# Autodesk Inventor assembly: SKF_SYWK 30 YTH
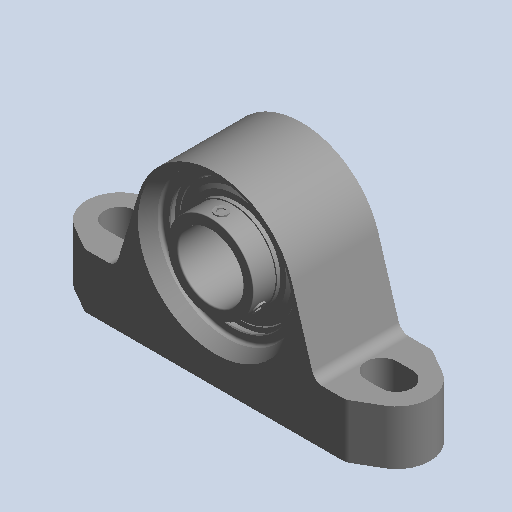
[picture p0: Inventor's stored thumbnail of the model, 512x512]
Saved by Autodesk Inventor 2022.1 (Build 261234000, 234)
## iProperties
Category: PARTsolutions
Company: SKF
Part Number: SKF_SYWK 30 YTH
Catalog Web Link: www.cadenas.de
Description: AYP_001_HC_HH_HY-AYL_001_HP-Y-bearing plummer block units
Vendor: SKF
Document SubType Name: Assembly
Designer: partserver
Manufacturer: SKF
Mass: 431.299 g
Surface Area: 643.844 cm^2
Volume: 166.494 cm^3
Density: 2.59047 g/cm^3
PSOL_IDENT_0: {$CADENAS_DATA\23d-libs\skf\bearings_units_and_housings\bearing_units\ball_bearing_units\y-units\ayp
PSOL_IDENT_1: _001_hc_hh_hy-ayl_001_hp.prj},212 {VTYP=3D},{STYP=ASSTAB},{NB=SKF_SYWK 30 YTH},{LINA=SKF_SYWK 30 YTH
PSOL_IDENT_2: },{NN=AYP_001_HC_HH_HY-AYL_001_HP},{DATE=17.09.2021 07:33:22},{GEOMDATE=07.09.2021 05:49:17},{VERSIO
PSOL_IDENT_3: N=},{LINEID=6610},{WBVAR=COVER},{WBNUMERIC=}  {NB=SKF_SYWK 30 YTH},{LINA=SKF_SYWK 30 YTH},{KT=DUMMY}
PSOL_IDENT_4: ,{DESIGNATION=SYWK 30 YTH},{COVER=},{DDALG=30.0000},{DD=30},{DDX=},{DD1=39.7},{DD2=},{DAA=},{HA=},{A=
PSOL_IDENT_5: MIN},{AX=40},{AXX=},{AXXX=},{A1=MIN},{A1X=25},{A1XX=},{A1XXX=},{A5=MIN},{A5X=30.5},{A5XX=},{B=38.100
PSOL_IDENT_6: },{B1=38.100},{B1X=},{B4ALG=5.000},{B4=5},{B4X=},{H=},{HX=82},{HXX=},{HXXX=},{H1=},{H1X=42.9},{H1XX=
PSOL_IDENT_7: },{H1XXX=},{H2=},{H2X=19},{H2XX=},{H2XXX=},{J=},{JX=121},{JXX=},{JXXX=},{JMAX=},{JMAXX=128},{JMAXXX=
PSOL_IDENT_8: },{JMIN=},{JMINX=114},{JMINXX=},{L=},{LX=159},{LXX=},{LXXX=},{N=},{NX=21.5},{NXX=},{NXXX=},{N1=},{N1
PSOL_IDENT_9: X=14.5},{N1XX=},{N1XXX=},{SS1=},{SS1X=22.2},{RG=},{RGX=},{R1=},{R1X=},{RALPHA=},{RALPHAX=},{DN=},{SW
PSOL_IDENT_10: N=},{GN=},{J6=},{J7=},{D=62},{D1=62},{C=18},{R12=0.6},{B3=},{DW=9.525},{PITCH=46.000},{LOAD1=16.3},{
PSOL_IDENT_11: LOAD2=11.2},{LOAD3=0.475},{SPEED1=3800},{II=1},{Z=9},{MASS=},{MASSX=0.52},{MASSXX=},{G2=M6x0.75},{HK
PSOL_IDENT_12: SGS=3},{RTTGS=4},{AS=},{ALPHA=},{G=},{GX=12},{GXX=},{GXXX=},{GIN=},{GINX=0.5000000033},{GINXX=},{GIN
PSOL_IDENT_13: XXX=},{HOUSING=},{HOUSINGX=SYWK 506 Y},{HOUSINGXX=},{HOUSINGXXX=},{BEARING=YAR 206-2RF/HV},{BEARINGX=
PSOL_IDENT_14: },{SLEEVE=},{BS=},{RING=},{ECALG=ECW 206},{EC=},{ECX=},{ECXX=},{ECXXX=ECW 206},{POPULAR=},{PPATH=y-b
PSOL_IDENT_15: earing_plummer_block_units_parts/ayp_001_hc_hh_hy-ayl_001_hp_asmtpl.prj},{COVERALG=  '', 'No end cov
PSOL_IDENT_16: er', 'ECW 206', 'ECW 206' },{SUPPRESSED=unsuppressed},{DESIGN=syk},{TC=SYWK 30 YTH}
NB: SKF_SYWK 30 YTH
NN: AYP_001_HC_HH_HY-AYL_001_HP
NT: Y-bearing plummer block units
NBSYN: SKF_$TC.
LINA: SKF_SYWK 30 YTH
CATALOG: SKF
DESIGNATION: SYWK 30 YTH
COVER: No end cover
DDALG: 30
DD1: 39.7
A: 0
A1: 0
A5: 0
B: 38.1
B1: 38.1
B4ALG: 5
LOAD1: 16.3
LOAD2: 11.2
LOAD3: 0.475
SPEED1: 3800
G2: M6x0.75
HKSGS: 3
RTTGS: 4
BEARING: YAR 206-2RF/HV
SUPPRESSED: unsuppressed
SUPPLIER: SKF
ARTICLENO: SKF_SYWK 30 YTH
BOMINFO: SKF_SYWK 30 YTH
CREATOR: CADENAS GmbH
Title: SKF_SYWK 30 YTH
Author: Cadenas PARTsolutions
Comments: Y-bearing plummer block units
## Documents named in this file (4)
- C:\Users\seb_0\Desktop\PDM\ProyectoRobotPallet\Soportes\Rodamiento con soporte de pie\SKF_SYWK 30 YTH.iam
- C:\Users\seb_0\Desktop\PDM\ProyectoRobotPallet\Soportes\Rodamiento con soporte de pie\housingSYWK 506 Y-h.ipt
- C:\Users\seb_0\Desktop\PDM\ProyectoRobotPallet\Soportes\Rodamiento con soporte de pie\YAR 206-2RF_HV-39_7103004206-b.ipt
- C:\Users\seb_0\Desktop\PDM\ProyectoRobotPallet\Soportes\Rodamiento con soporte de pie\30-62-38_1-18-ybrg1-619_525-46-b.ipt
## Components (11 placed, 3 different names)
1. housingSYWK 506 Y-h:1
2. YAR 206-2RF_HV-39_7103004206-b:1 — ball_1_XY@2 <-> ball_XY@3, ball_1_Z@2 <-> ball_Z@3, ball_1_YZ@2 <-> ball_YZ@3, ball_2_XY@2 <-> ball_XY@4, ball_2_Z@2 <-> ball_Z@4, ball_2_YZ@2 <-> ball_YZ@4, ball_3_XY@2 <-> ball_XY@5, ball_3_Z@2 <-> ball_Z@5, ball_3_YZ@2 <-> ball_YZ@5, ball_4_XY@2 <-> ball_XY@6, ball_4_Z@2 <-> ball_Z@6, ball_4_YZ@2 <-> ball_YZ@6, ball_5_XY@2 <-> ball_XY@7, ball_5_Z@2 <-> ball_Z@7, ball_5_YZ@2 <-> ball_YZ@7, ball_6_XY@2 <-> ball_XY@8, ball_6_Z@2 <-> ball_Z@8, ball_6_YZ@2 <-> ball_YZ@8, ball_7_XY@2 <-> ball_XY@9, ball_7_Z@2 <-> ball_Z@9, ball_7_YZ@2 <-> ball_YZ@9, ball_8_XY@2 <-> ball_XY@10, ball_8_Z@2 <-> ball_Z@10, ball_8_YZ@2 <-> ball_YZ@10, ball_9_XY@2 <-> ball_XY@11, ball_9_Z@2 <-> ball_Z@11, ball_9_YZ@2 <-> ball_YZ@11
3. 30-62-38_1-18-ybrg1-619_525-46-b:1 — ball_1_XY@2 <-> ball_XY@3, ball_1_Z@2 <-> ball_Z@3, ball_1_YZ@2 <-> ball_YZ@3
4. 30-62-38_1-18-ybrg1-619_525-46-b:2 — ball_2_XY@2 <-> ball_XY@4, ball_2_Z@2 <-> ball_Z@4, ball_2_YZ@2 <-> ball_YZ@4
5. 30-62-38_1-18-ybrg1-619_525-46-b:3 — ball_3_XY@2 <-> ball_XY@5, ball_3_Z@2 <-> ball_Z@5, ball_3_YZ@2 <-> ball_YZ@5
6. 30-62-38_1-18-ybrg1-619_525-46-b:4 — ball_4_XY@2 <-> ball_XY@6, ball_4_Z@2 <-> ball_Z@6, ball_4_YZ@2 <-> ball_YZ@6
7. 30-62-38_1-18-ybrg1-619_525-46-b:5 — ball_5_XY@2 <-> ball_XY@7, ball_5_Z@2 <-> ball_Z@7, ball_5_YZ@2 <-> ball_YZ@7
8. 30-62-38_1-18-ybrg1-619_525-46-b:6 — ball_6_XY@2 <-> ball_XY@8, ball_6_Z@2 <-> ball_Z@8, ball_6_YZ@2 <-> ball_YZ@8
9. 30-62-38_1-18-ybrg1-619_525-46-b:7 — ball_7_XY@2 <-> ball_XY@9, ball_7_Z@2 <-> ball_Z@9, ball_7_YZ@2 <-> ball_YZ@9
10. 30-62-38_1-18-ybrg1-619_525-46-b:8 — ball_8_XY@2 <-> ball_XY@10, ball_8_Z@2 <-> ball_Z@10, ball_8_YZ@2 <-> ball_YZ@10
11. 30-62-38_1-18-ybrg1-619_525-46-b:9 — ball_9_XY@2 <-> ball_XY@11, ball_9_Z@2 <-> ball_Z@11, ball_9_YZ@2 <-> ball_YZ@11
## Relationships (27: Mate 18, Angle 9)
- ball_1_XY@2 <-> ball_XY@3 [Mate]: YAR 206-2RF_HV-39_7103004206-b:1 ↔ 30-62-38_1-18-ybrg1-619_525-46-b:1
- ball_1_Z@2 <-> ball_Z@3 [Mate]: YAR 206-2RF_HV-39_7103004206-b:1 ↔ 30-62-38_1-18-ybrg1-619_525-46-b:1
- ball_1_YZ@2 <-> ball_YZ@3 [Angle] (0 deg): YAR 206-2RF_HV-39_7103004206-b:1 ↔ 30-62-38_1-18-ybrg1-619_525-46-b:1
- ball_2_XY@2 <-> ball_XY@4 [Mate]: YAR 206-2RF_HV-39_7103004206-b:1 ↔ 30-62-38_1-18-ybrg1-619_525-46-b:2
- ball_2_Z@2 <-> ball_Z@4 [Mate]: YAR 206-2RF_HV-39_7103004206-b:1 ↔ 30-62-38_1-18-ybrg1-619_525-46-b:2
- ball_2_YZ@2 <-> ball_YZ@4 [Angle] (0 deg): YAR 206-2RF_HV-39_7103004206-b:1 ↔ 30-62-38_1-18-ybrg1-619_525-46-b:2
- ball_3_XY@2 <-> ball_XY@5 [Mate]: YAR 206-2RF_HV-39_7103004206-b:1 ↔ 30-62-38_1-18-ybrg1-619_525-46-b:3
- ball_3_Z@2 <-> ball_Z@5 [Mate]: YAR 206-2RF_HV-39_7103004206-b:1 ↔ 30-62-38_1-18-ybrg1-619_525-46-b:3
- ball_3_YZ@2 <-> ball_YZ@5 [Angle] (0 deg): YAR 206-2RF_HV-39_7103004206-b:1 ↔ 30-62-38_1-18-ybrg1-619_525-46-b:3
- ball_4_XY@2 <-> ball_XY@6 [Mate]: YAR 206-2RF_HV-39_7103004206-b:1 ↔ 30-62-38_1-18-ybrg1-619_525-46-b:4
- ball_4_Z@2 <-> ball_Z@6 [Mate]: YAR 206-2RF_HV-39_7103004206-b:1 ↔ 30-62-38_1-18-ybrg1-619_525-46-b:4
- ball_4_YZ@2 <-> ball_YZ@6 [Angle] (0 deg): YAR 206-2RF_HV-39_7103004206-b:1 ↔ 30-62-38_1-18-ybrg1-619_525-46-b:4
- ball_5_XY@2 <-> ball_XY@7 [Mate]: YAR 206-2RF_HV-39_7103004206-b:1 ↔ 30-62-38_1-18-ybrg1-619_525-46-b:5
- ball_5_Z@2 <-> ball_Z@7 [Mate]: YAR 206-2RF_HV-39_7103004206-b:1 ↔ 30-62-38_1-18-ybrg1-619_525-46-b:5
- ball_5_YZ@2 <-> ball_YZ@7 [Angle] (0 deg): YAR 206-2RF_HV-39_7103004206-b:1 ↔ 30-62-38_1-18-ybrg1-619_525-46-b:5
- ball_6_XY@2 <-> ball_XY@8 [Mate]: YAR 206-2RF_HV-39_7103004206-b:1 ↔ 30-62-38_1-18-ybrg1-619_525-46-b:6
- ball_6_Z@2 <-> ball_Z@8 [Mate]: YAR 206-2RF_HV-39_7103004206-b:1 ↔ 30-62-38_1-18-ybrg1-619_525-46-b:6
- ball_6_YZ@2 <-> ball_YZ@8 [Angle] (0 deg): YAR 206-2RF_HV-39_7103004206-b:1 ↔ 30-62-38_1-18-ybrg1-619_525-46-b:6
- ball_7_XY@2 <-> ball_XY@9 [Mate]: YAR 206-2RF_HV-39_7103004206-b:1 ↔ 30-62-38_1-18-ybrg1-619_525-46-b:7
- ball_7_Z@2 <-> ball_Z@9 [Mate]: YAR 206-2RF_HV-39_7103004206-b:1 ↔ 30-62-38_1-18-ybrg1-619_525-46-b:7
- ball_7_YZ@2 <-> ball_YZ@9 [Angle] (0 deg): YAR 206-2RF_HV-39_7103004206-b:1 ↔ 30-62-38_1-18-ybrg1-619_525-46-b:7
- ball_8_XY@2 <-> ball_XY@10 [Mate]: YAR 206-2RF_HV-39_7103004206-b:1 ↔ 30-62-38_1-18-ybrg1-619_525-46-b:8
- ball_8_Z@2 <-> ball_Z@10 [Mate]: YAR 206-2RF_HV-39_7103004206-b:1 ↔ 30-62-38_1-18-ybrg1-619_525-46-b:8
- ball_8_YZ@2 <-> ball_YZ@10 [Angle] (0 deg): YAR 206-2RF_HV-39_7103004206-b:1 ↔ 30-62-38_1-18-ybrg1-619_525-46-b:8
- ball_9_XY@2 <-> ball_XY@11 [Mate]: YAR 206-2RF_HV-39_7103004206-b:1 ↔ 30-62-38_1-18-ybrg1-619_525-46-b:9
- ball_9_Z@2 <-> ball_Z@11 [Mate]: YAR 206-2RF_HV-39_7103004206-b:1 ↔ 30-62-38_1-18-ybrg1-619_525-46-b:9
- ball_9_YZ@2 <-> ball_YZ@11 [Angle] (0 deg): YAR 206-2RF_HV-39_7103004206-b:1 ↔ 30-62-38_1-18-ybrg1-619_525-46-b:9
